# Autodesk Inventor assembly: Lady Brown HS Axle
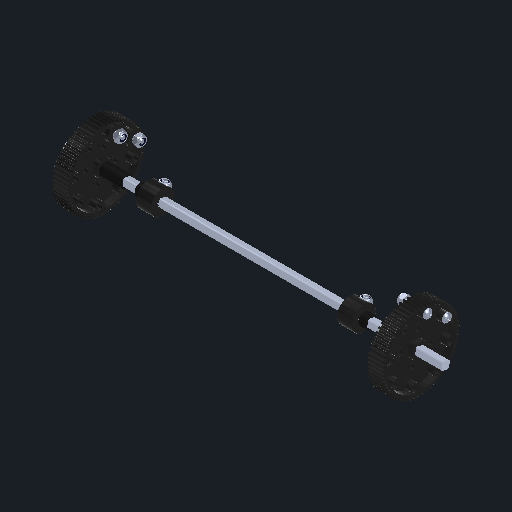
[picture p0: Inventor's stored thumbnail of the model, 512x512]
Saved by Autodesk Inventor 2025 (Build 290162000, 162)
## iProperties
Created: 2024-12-19
Part Number: Lady Brown HS Axle
Document SubType Name: Assembly
Designer: Juan
Author: Juan
## Documents named in this file (14)
- C:\Users\Juan\Documents\GitHub\ATUM-VRC-High-Stakes-CAD\Protobot\Lady Brown HS Axle.iam
- C:\Users\Juan\Documents\GitHub\ATUM-VRC-High-Stakes-CAD\VEX-CAD-Inventor\Motion\Shaft HS\Shaft HS\Shaft HS 12.5 in.ipt
- C:\Users\Juan\Documents\GitHub\ATUM-VRC-High-Stakes-CAD\VEX-CAD-Inventor\Motion\Shaft HS\Shaft HS.ipt
- C:\Users\Juan\Documents\GitHub\ATUM-VRC-High-Stakes-CAD\VEX-CAD-Inventor\Motion\Shaft HS\HS Spacer\HSpacer .5000.ipt
- C:\Users\Juan\Documents\GitHub\ATUM-VRC-High-Stakes-CAD\VEX-CAD-Inventor\Motion\Shaft HS\HS Spacer.ipt
- C:\Users\Juan\Documents\GitHub\ATUM-VRC-High-Stakes-CAD\VEX-CAD-Inventor\Motion\Shaft HS\HS Spacer\HSpacer .2500.ipt
- C:\Users\Juan\Documents\GitHub\ATUM-VRC-High-Stakes-CAD\60T High Strength Gear (276-5035)\60T High Strength Gear (276-5035).ipt
- C:\Users\Juan\Documents\GitHub\ATUM-VRC-High-Stakes-CAD\VEX-CAD-Inventor\Motion\Spacers\Spacer Nylon .500 OD\NSpacer Black .500 OD x .125.ipt
- C:\Users\Juan\Documents\GitHub\ATUM-VRC-High-Stakes-CAD\VEX-CAD-Inventor\Motion\Spacers\Spacer Nylon .500 OD.ipt
- C:\Users\Juan\Documents\GitHub\ATUM-VRC-High-Stakes-CAD\VEX-CAD-Inventor\Motion\Shaft HS\HS Shaft Collar.ipt
- C:\Users\Juan\Documents\GitHub\ATUM-VRC-High-Stakes-CAD\VEX-CAD-Inventor\Structure\Hardware\Screw Steel - Star\SScrew Star Smooth .625.ipt
- C:\Users\Juan\Documents\GitHub\ATUM-VRC-High-Stakes-CAD\VEX-CAD-Inventor\Structure\Hardware\Screw Steel - Star.ipt
- C:\Users\Juan\Documents\GitHub\ATUM-VRC-High-Stakes-CAD\VEX-CAD-Inventor\Structure\Hardware\Nut Thin Nylock.ipt
- C:\Users\Juan\Documents\GitHub\ATUM-VRC-High-Stakes-CAD\VEX-CAD-Inventor\Structure\Hardware\Screw Steel - Star\SScrew Star Smooth .875.ipt
## Components (25 placed, 9 different names)
1. Shaft HS 12.5 in:1
2. HSpacer .5000:1
3. HSpacer .5000:2
4. HSpacer .2500:3
5. 60T High Strength Gear (276-5035):1
6. 60T High Strength Gear (276-5035):2
7. HSpacer .2500:4
8. NSpacer Black .500 OD x .125:1
9. NSpacer Black .500 OD x .125:2
10. HS Shaft Collar:1
11. HS Shaft Collar:2
12. HSpacer .2500:5
13. HSpacer .2500:6
14. SScrew Star Smooth .625:1
15. Nut Thin Nylock:1
16. SScrew Star Smooth .625:2
17. Nut Thin Nylock:2
18. SScrew Star Smooth .875:3
19. SScrew Star Smooth .875:4
20. Nut Thin Nylock:3
21. Nut Thin Nylock:4
22. Nut Thin Nylock:5
23. Nut Thin Nylock:6
24. SScrew Star Smooth .875:5
25. SScrew Star Smooth .875:6
## Relationships (45: Mate 39, WeldJoint 6)
- [Mate]: Shaft HS 12.5 in:1 ↔ HSpacer .5000:2
- [Mate]: Shaft HS 12.5 in:1 ↔ HSpacer .5000:2
- [Mate]: Shaft HS 12.5 in:1 ↔ HSpacer .2500:3
- [Mate]: Shaft HS 12.5 in:1 ↔ HSpacer .2500:3
- [Mate]: HSpacer .5000:2 ↔ HSpacer .2500:3
- [Mate]: Shaft HS 12.5 in:1 ↔ HSpacer .5000:1
- [Mate]: Shaft HS 12.5 in:1 ↔ HSpacer .5000:1
- [Mate]: Shaft HS 12.5 in:1 ↔ 60T High Strength Gear (276-5035):2
- [Mate]: Shaft HS 12.5 in:1 ↔ 60T High Strength Gear (276-5035):2
- [Mate]: Shaft HS 12.5 in:1 ↔ 60T High Strength Gear (276-5035):1
- [Mate]: Shaft HS 12.5 in:1 ↔ 60T High Strength Gear (276-5035):1
- [Mate]: HSpacer .2500:3 ↔ 60T High Strength Gear (276-5035):1
- [Mate]: Shaft HS 12.5 in:1 ↔ HSpacer .2500:4
- [Mate]: Shaft HS 12.5 in:1 ↔ HSpacer .2500:4
- [Mate]: HSpacer .5000:1 ↔ HSpacer .2500:4
- [Mate]: 60T High Strength Gear (276-5035):2 ↔ HSpacer .2500:4
- [Mate]: 60T High Strength Gear (276-5035):2 ↔ NSpacer Black .500 OD x .125:1
- [Mate]: 60T High Strength Gear (276-5035):2 ↔ NSpacer Black .500 OD x .125:1
- [Mate]: 60T High Strength Gear (276-5035):2 ↔ NSpacer Black .500 OD x .125:2
- [Mate]: 60T High Strength Gear (276-5035):2 ↔ NSpacer Black .500 OD x .125:2
- [Mate]: Shaft HS 12.5 in:1 ↔ HS Shaft Collar:1
- [Mate]: Shaft HS 12.5 in:1 ↔ HS Shaft Collar:1
- [Mate]: Shaft HS 12.5 in:1 ↔ HS Shaft Collar:2
- [Mate]: Shaft HS 12.5 in:1 ↔ HS Shaft Collar:2
- [Mate]: Shaft HS 12.5 in:1 ↔ HSpacer .2500:5
- [Mate]: Shaft HS 12.5 in:1 ↔ HSpacer .2500:5
- [Mate]: HS Shaft Collar:1 ↔ HSpacer .2500:5
- [Mate]: Shaft HS 12.5 in:1 ↔ HSpacer .2500:6
- [Mate]: Shaft HS 12.5 in:1 ↔ HSpacer .2500:6
- [Mate]: HS Shaft Collar:2 ↔ HSpacer .2500:6
- [Mate]: HS Shaft Collar:1 ↔ SScrew Star Smooth .625:1
- [Mate]: HS Shaft Collar:1 ↔ SScrew Star Smooth .625:1
- [Mate]: SScrew Star Smooth .625:1 ↔ Nut Thin Nylock:1
- [Mate]: HS Shaft Collar:1 ↔ Nut Thin Nylock:1
- [Mate]: SScrew Star Smooth .625:2 ↔ Nut Thin Nylock:2
- [Mate]: HS Shaft Collar:2 ↔ SScrew Star Smooth .625:2
- [Mate]: HS Shaft Collar:2 ↔ SScrew Star Smooth .625:2
- [Mate]: SScrew Star Smooth .625:2 ↔ Nut Thin Nylock:2
- [Mate]: HS Shaft Collar:2 ↔ Nut Thin Nylock:2
- [WeldJoint]: 60T High Strength Gear (276-5035):1 ↔ SScrew Star Smooth .875:3
- [WeldJoint]: 60T High Strength Gear (276-5035):1 ↔ SScrew Star Smooth .875:4
- [WeldJoint] (-4.1656 mm): SScrew Star Smooth .875:4 ↔ Nut Thin Nylock:4
- [WeldJoint]: 60T High Strength Gear (276-5035):2 ↔ SScrew Star Smooth .875:6
- [WeldJoint]: 60T High Strength Gear (276-5035):2 ↔ SScrew Star Smooth .875:5
- [WeldJoint] (-4.5212 mm): Nut Thin Nylock:6 ↔ SScrew Star Smooth .875:5
## Named parameters: d1724_d1722 = 0 mm
